# Autodesk Inventor assembly: Housing_Assembly
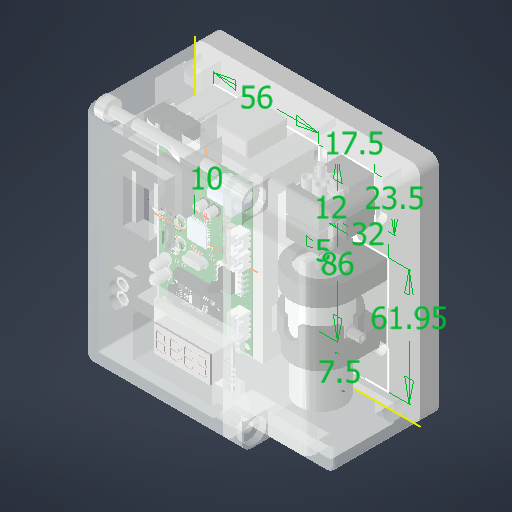
[picture p0: Inventor's stored thumbnail of the model, 512x512]
Saved by Autodesk Inventor 2026.2 (Build 302298000, 298)
## iProperties
Created: 2026-02-03
Part Number: Housing_Assembly
Document SubType Name: Assembly
Designer: vckot
Author: vckot
## Documents named in this file (12)
- C:\Users\vckot\OneDrive\Documents\Vaibhav\capstone\CAD_files\Housing_Assembly.iam
- C:\Users\vckot\OneDrive\Documents\Vaibhav\capstone\CAD_files\PCB_Housing\TourniquetPCBV1_Updated\TourniquetPCBV1_Updated\TourniquetPCBV1_Updated.iam
- C:\Users\vckot\OneDrive\Documents\Vaibhav\capstone\CAD_files\Batteries\Battery_Small.ipt
- C:\Users\vckot\OneDrive\Documents\Vaibhav\capstone\CAD_files\PCB_Housing\PCB_Housing_01_001.ipt
- C:\Users\vckot\OneDrive\Documents\Vaibhav\capstone\CAD_files\Motor\Motor_Assembly.iam
- C:\Users\vckot\OneDrive\Documents\Vaibhav\capstone\CAD_files\Motor_Valve\Motor_Valve_Assembly.iam
- C:\Users\vckot\OneDrive\Documents\Vaibhav\capstone\CAD_files\Batteries\Battery_Large.ipt
- C:\Users\vckot\OneDrive\Documents\Vaibhav\capstone\CAD_files\PCB_Housing\PCB_Housing_01_002.ipt
- C:\Users\vckot\OneDrive\Documents\Vaibhav\capstone\CAD_files\PCB_Housing\PCB_Housing_01_003.ipt
- C:\Users\vckot\OneDrive\Documents\Vaibhav\capstone\CAD_files\7_Segment_Display\Display TM1637.ipt
- C:\Users\vckot\OneDrive\Documents\Vaibhav\capstone\CAD_files\Snap_Switch\Snap_Switch_Assembly.iam
- C:\Users\vckot\OneDrive\Documents\Vaibhav\capstone\CAD_files\PCB_Housing\PCB_Housing_01_004.ipt
## Components (11 placed, 11 different names)
1. TourniquetPCBV1_Updated:1 [sub-assembly] — Mate:1, Mate:2, Flush:1, Mate:3, Mate:4, Mate:6, Flush:6
2. Battery_Small:1 — Mate:1, Mate:2, Flush:1, Flush:2, Mate:5
3. PCB_Housing_01_001:1 — Mate:3, Mate:4, Flush:2, Mate:9, Mate:11, Mate:12
4. Motor_Assembly:1 [sub-assembly] — Mate:13, Mate:19, Mate:20
5. Motor_Valve_Assembly:1 [sub-assembly] — Mate:16, Mate:21, Mate:22
6. Battery_Large:1 — Mate:5, Mate:6, Flush:6
7. PCB_Housing_01_002:1 — Mate:23, Flush:11, Mate:24, Mate:25, Mate:26, Mate:27, Mate:28, Mate:29, Flush:12, Flush:13
8. PCB_Housing_01_003:1 — Mate:9, Flush:8, Mate:10, Mate:11, Mate:12, Flush:9, Mate:13, Mate:16, Mate:19, Mate:20, Mate:21, Mate:22, Mate:23, Flush:11, Flush:12, Flush:14, Flush:15
9. Display TM1637:1 — Mate:24, Mate:25, Mate:26
10. Snap_Switch_Assembly:1 [sub-assembly] — Mate:27, Mate:28, Mate:29
11. PCB_Housing_01_004:1 — Flush:13, Flush:14, Flush:15
## Relationships (33: Mate 23, Flush 10)
- Mate:1 (10 mm): TourniquetPCBV1_Updated:1 ↔ Battery_Small:1
- Mate:2: TourniquetPCBV1_Updated:1 ↔ Battery_Small:1
- Flush:1: TourniquetPCBV1_Updated:1 ↔ Battery_Small:1
- Mate:3: TourniquetPCBV1_Updated:1 ↔ PCB_Housing_01_001:1
- Mate:4: TourniquetPCBV1_Updated:1 ↔ PCB_Housing_01_001:1
- Flush:2: Battery_Small:1 ↔ PCB_Housing_01_001:1
- Mate:5: Battery_Small:1 ↔ Battery_Large:1
- Mate:6: TourniquetPCBV1_Updated:1 ↔ Battery_Large:1
- Flush:6: TourniquetPCBV1_Updated:1 ↔ Battery_Large:1
- Mate:9: PCB_Housing_01_001:1 ↔ PCB_Housing_01_003:1
- Flush:8: PCB_Housing_01_003:1
- Mate:10: PCB_Housing_01_003:1
- Mate:11: PCB_Housing_01_001:1 ↔ PCB_Housing_01_003:1
- Mate:12: PCB_Housing_01_001:1 ↔ PCB_Housing_01_003:1
- Flush:9: PCB_Housing_01_003:1
- Mate:13: Motor_Assembly:1 ↔ PCB_Housing_01_003:1
- Mate:16: Motor_Valve_Assembly:1 ↔ PCB_Housing_01_003:1
- Mate:19: Motor_Assembly:1 ↔ PCB_Housing_01_003:1
- Mate:20: Motor_Assembly:1 ↔ PCB_Housing_01_003:1
- Mate:21: Motor_Valve_Assembly:1 ↔ PCB_Housing_01_003:1
- Mate:22: Motor_Valve_Assembly:1 ↔ PCB_Housing_01_003:1
- Mate:23: PCB_Housing_01_002:1 ↔ PCB_Housing_01_003:1
- Flush:11: PCB_Housing_01_002:1 ↔ PCB_Housing_01_003:1
- Mate:24: PCB_Housing_01_002:1 ↔ Display TM1637:1
- Mate:25: PCB_Housing_01_002:1 ↔ Display TM1637:1
- Mate:26: PCB_Housing_01_002:1 ↔ Display TM1637:1
- Mate:27: PCB_Housing_01_002:1 ↔ Snap_Switch_Assembly:1
- Mate:28: PCB_Housing_01_002:1 ↔ Snap_Switch_Assembly:1
- Mate:29: PCB_Housing_01_002:1 ↔ Snap_Switch_Assembly:1
- Flush:12: PCB_Housing_01_002:1 ↔ PCB_Housing_01_003:1
- Flush:13: PCB_Housing_01_002:1 ↔ PCB_Housing_01_004:1
- Flush:14: PCB_Housing_01_003:1 ↔ PCB_Housing_01_004:1
- Flush:15: PCB_Housing_01_003:1 ↔ PCB_Housing_01_004:1
